# Autodesk Inventor assembly: Mesa_Montagem_001
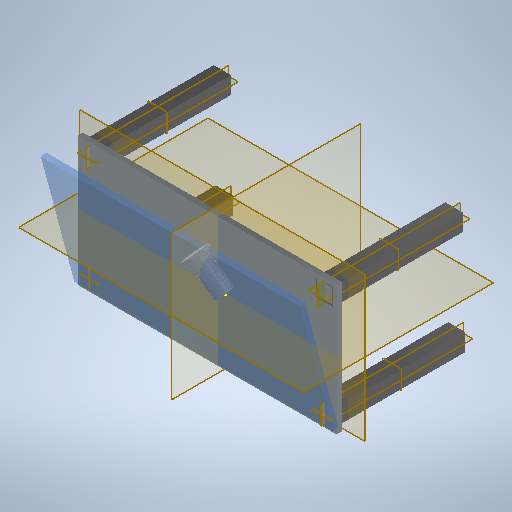
[picture p0: Inventor's stored thumbnail of the model, 512x512]
Saved by Autodesk Inventor 2025.2 (Build 292293000, 293)
## iProperties
Created: 2025-04-07
Part Number: Mesa_Montagem_001
Document SubType Name: Assembly
Designer: ishad
Author: ishad
## Documents named in this file (4)
- C:\Users\ishad\Documents\Inventor\Sessao_10_4_7_2025\Mesa_Montagem_001.iam
- C:\Users\ishad\Documents\Inventor\Sessao_10_4_7_2025\Mesa_001_0001.ipt
- C:\Users\ishad\Documents\Inventor\Sessao_10_4_7_2025\Perna_001_0001.ipt
- C:\Users\ishad\Documents\Inventor\Sessao_4_25_03_2025\Coil.ipt
## Components (7 placed, 3 different names)
1. Mesa_001_0001:1 — Flush:1, Flush:2, Flush:3, Flush:4, Flush:6, Flush:7, Flush:8, Flush:9, Flush:10, Flush:11, Mate:1, Flush:12, Flush:13, Angle:1
2. Perna_001_0001:1 — Flush:4, Flush:6, Flush:7
3. Perna_001_0001:2 — Flush:10, Flush:11
4. Perna_001_0001:3 — Mate:1, Flush:12, Flush:13
5. Perna_001_0001:4 — Flush:8, Flush:9
6. Coil:1 — Tangent:1
7. Mesa_001_0001:2 — Angle:1
## Relationships (15: Flush 12, Mate 1, Tangent 1, Angle 1)
- Flush:1 (-59.971 mm): Mesa_001_0001:1
- Flush:2 (-10.54 mm): Mesa_001_0001:1
- Flush:3 (55.51 mm): Mesa_001_0001:1
- Flush:4: Mesa_001_0001:1 ↔ Perna_001_0001:1
- Flush:6 (20 mm): Mesa_001_0001:1 ↔ Perna_001_0001:1
- Flush:7 (20 mm): Mesa_001_0001:1 ↔ Perna_001_0001:1
- Flush:8 (20 mm): Mesa_001_0001:1 ↔ Perna_001_0001:4
- Flush:9 (20 mm): Mesa_001_0001:1 ↔ Perna_001_0001:4
- Flush:10 (20 mm): Mesa_001_0001:1 ↔ Perna_001_0001:2
- Flush:11 (20 mm): Mesa_001_0001:1 ↔ Perna_001_0001:2
- Mate:1: Mesa_001_0001:1 ↔ Perna_001_0001:3
- Flush:12 (20 mm): Mesa_001_0001:1 ↔ Perna_001_0001:3
- Flush:13 (20 mm): Mesa_001_0001:1 ↔ Perna_001_0001:3
- Tangent:1 (20 mm): Coil:1
- Angle:1 (165 deg): Mesa_001_0001:1 ↔ Mesa_001_0001:2
